# Autodesk Inventor assembly: uMule-Koło
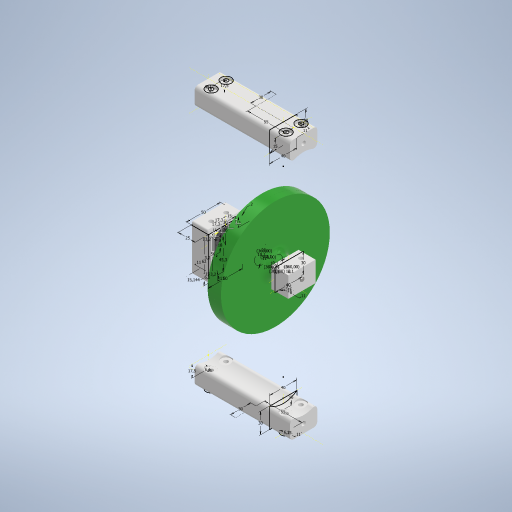
[picture p0: Inventor's stored thumbnail of the model, 512x512]
Saved by Autodesk Inventor 2024.2 (Build 282272000, 272)
## iProperties
Created: 2024-10-21
Part Number: uMule-Koło
Document SubType Name: Assembly
Designer: owozn
Author: owozn
## Documents named in this file (7)
- C:\Users\owozn\Documents\Semestr 7\Inżynierka\Modele 3D\uMule-Koło.iam
- C:\Users\owozn\Documents\Semestr 7\Inżynierka\Modele 3D\uMule-kolo_napędowe.ipt
- C:\Users\owozn\Documents\Semestr 7\Inżynierka\Modele 3D\rx64H\rx64H.ipt
- C:\Users\owozn\Documents\Inventor\Content Center Files\R2024\pl-PL\ANSI B18.2.3.5M\ANSI B18.2.3.5M - M6 x 1 x 60.ipt
- C:\Users\owozn\Documents\Semestr 7\Inżynierka\Modele 3D\uMule-Uchwyt_koła.ipt
- C:\Users\owozn\Documents\Semestr 7\Inżynierka\Modele 3D\uMule-ogranicznik_koła.ipt
- C:\Users\owozn\Documents\Semestr 7\Inżynierka\Modele 3D\uMule-uchwyt_dx_góra.ipt
## Components (8 placed, 6 different names)
1. uMule-kolo_napędowe:1 — Zestawiające:1, Zestawiające:2, Zestawiające:3, Zestawiające:4, Zestawiające:7
2. uMule-kolo_napędowe:2 — Zestawiające:1, Zestawiające:2, Zestawiające:3, Zestawiające:5, Wstawiające:1
3. rx64H:1 — Zestawiające:4, Zestawiające:5, Równoległe:2, Zestawiające:15, Zestawiające:16
4. Śruba z łbem sześciokątnym - Metryczny M6 x 1 x 60:1 — Wstawiające:1, Zestawiające:6, Zestawiające:9
5. uMule-Uchwyt_koła:1 — Zestawiające:6, Zestawiające:7, Zestawiające:10, Równoległe:1
6. uMule-ogranicznik_koła:1 — Zestawiające:9, Zestawiające:10, Zestawiające:11, Zestawiające:12, Równoległe:3
7. uMule-ogranicznik_koła:2 — Zestawiające:11, Zestawiające:12, Równoległe:1
8. uMule-uchwyt_dx_góra:1 — Równoległe:2, Równoległe:3, Zestawiające:15, Zestawiające:16
## Relationships (17: Mate 13, Flush 3, Insert 1)
- Zestawiające:1 [Mate]: uMule-kolo_napędowe:1 ↔ uMule-kolo_napędowe:2
- Zestawiające:2 [Mate]: uMule-kolo_napędowe:1 ↔ uMule-kolo_napędowe:2
- Zestawiające:3 [Mate]: uMule-kolo_napędowe:1 ↔ uMule-kolo_napędowe:2
- Zestawiające:4 [Mate]: uMule-kolo_napędowe:1 ↔ rx64H:1
- Zestawiające:5 [Mate]: uMule-kolo_napędowe:2 ↔ rx64H:1
- Wstawiające:1 [Insert]: uMule-kolo_napędowe:2 ↔ Śruba z łbem sześciokątnym - Metryczny M6 x 1 x 60:1
- Zestawiające:6 [Mate]: Śruba z łbem sześciokątnym - Metryczny M6 x 1 x 60:1 ↔ uMule-Uchwyt_koła:1
- Zestawiające:7 [Mate] (4 mm): uMule-kolo_napędowe:1 ↔ uMule-Uchwyt_koła:1
- Zestawiające:9 [Mate] (130 mm): Śruba z łbem sześciokątnym - Metryczny M6 x 1 x 60:1 ↔ uMule-ogranicznik_koła:1
- Zestawiające:10 [Mate]: uMule-Uchwyt_koła:1 ↔ uMule-ogranicznik_koła:1
- Zestawiające:11 [Mate]: uMule-ogranicznik_koła:1 ↔ uMule-ogranicznik_koła:2
- Zestawiające:12 [Mate]: uMule-ogranicznik_koła:1 ↔ uMule-ogranicznik_koła:2
- Równoległe:1 [Flush] (180 mm): uMule-Uchwyt_koła:1 ↔ uMule-ogranicznik_koła:2
- Równoległe:2 [Flush]: rx64H:1 ↔ uMule-uchwyt_dx_góra:1
- Równoległe:3 [Flush] (168.662 mm): uMule-ogranicznik_koła:1 ↔ uMule-uchwyt_dx_góra:1
- Zestawiające:15 [Mate]: rx64H:1 ↔ uMule-uchwyt_dx_góra:1
- Zestawiające:16 [Mate]: rx64H:1 ↔ uMule-uchwyt_dx_góra:1
